# Autodesk Inventor assembly: HEXY
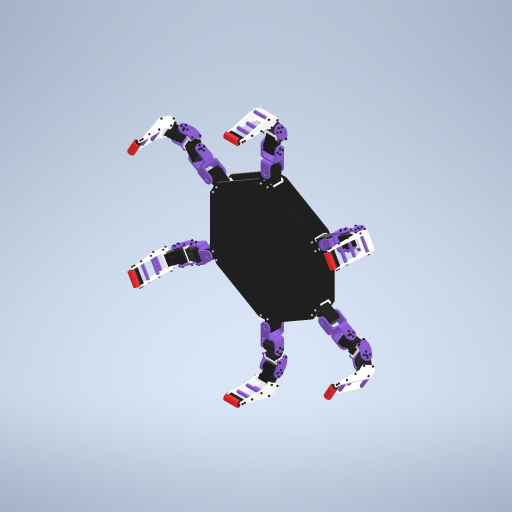
[picture p0: Inventor's stored thumbnail of the model, 512x512]
Saved by Autodesk Inventor 2024 (Build 280153000, 153)
## iProperties
Created: 2024-06-04
Part Number: HEXY
Document SubType Name: Assembly
Designer: Hemant
Author: Hemant
## Documents named in this file (3)
- C:\Users\Hemant\Desktop\Studies\MS Proj\V1\HEXY.iam
- C:\Users\Hemant\Desktop\Studies\MS Proj\V1\Body_Plate.ipt
- C:\Users\Hemant\Desktop\Studies\MS Proj\V1\Leg_assembly_V2.iam
## Components (8 placed, 2 different names)
1. Body_Plate:1 — Mate:1, Mate:2, Mate:3, Mate:4, Mate:5
2. Body_Plate:2 — Mate:4, Mate:5, Mate:6
3. Leg_assembly_V2:1 [sub-assembly] — Mate:1, Mate:2, Mate:3, Mate:6
4. Leg_assembly_V2:2 [sub-assembly]
5. Leg_assembly_V2:3 [sub-assembly]
6. Leg_assembly_V2:4 [sub-assembly]
7. Leg_assembly_V2:5 [sub-assembly]
8. Leg_assembly_V2:6 [sub-assembly]
## Component patterns: (6 elements, first: Leg_assembly_V2:1)
## Relationships (6: Mate 6)
- Mate:1: Body_Plate:1 ↔ Leg_assembly_V2:1
- Mate:2: Body_Plate:1 ↔ Leg_assembly_V2:1
- Mate:3: Body_Plate:1 ↔ Leg_assembly_V2:1
- Mate:4: Body_Plate:1 ↔ Body_Plate:2
- Mate:5: Body_Plate:1 ↔ Body_Plate:2
- Mate:6: Body_Plate:2 ↔ Leg_assembly_V2:1
